# Autodesk Inventor assembly: Lift - Main Drive Sprocket
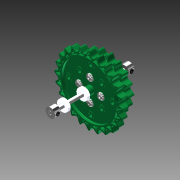
[picture p0: Inventor's stored thumbnail of the model, 180x180]
Saved by Autodesk Inventor 2012 (Build 160160000, 160)
## iProperties
Created: 2011-09-10
Part Number: Lift - Main Drive Sprocket
Document SubType Name: Assembly
Designer: Wade
Author: Wade
## Documents named in this file (9)
- C:\Users\Wade\Documents\1103 Robot - CAD Assembly\Lift - Main Drive Sprocket.iam
- C:\Users\Wade\Documents\24C VEX CAD Files\Drive Shafts\Drive Shaft (Square Bar) 3.625''.ipt
- C:\Users\Wade\Documents\24C VEX CAD Files\Gears & Pulleys\High Strength 24-Tooth Sprocket.ipt
- C:\Users\Wade\Documents\24C VEX CAD Files\Gears & Pulleys\High Strength 18-Tooth Sprocket.ipt
- C:\Users\Wade\Documents\1103 Robot - CAD Assembly\BEAM-0500.ipt
- C:\Users\Wade\Documents\24C VEX CAD Files\Other Parts\Shaft Collar (with Set Screw Installed).ipt
- C:\Users\Wade\Documents\24C VEX CAD Files\Washers & Spacers\Spacer (Nylon), 0.125''.ipt
- C:\Users\Wade\Documents\24C VEX CAD Files\Washers & Spacers\Spacer (Nylon), 0.250''.ipt
- C:\Users\Wade\Documents\24C VEX CAD Files\Screws & Nuts\Screw 8-32 x 0.375''-Silver.ipt
## Components (20 placed, 8 different names)
1. Drive Shaft (Square Bar) 3.625'':1 — Mate:1, Mate:2, Flush:1, Flush:2, Flush:4
2. High Strength 24-Tooth Sprocket:1 — Mate:1, Mate:2, Mate:3, Mate:4, Mate:5, Mate:6, Mate:7, Mate:8, Mate:9, Mate:10, Mate:11, Mate:22, Mate:23, Mate:24, Mate:25, Mate:26, Mate:27, Mate:28, Mate:29, Mate:31, Mate:33, Mate:35, Mate:36, Mate:37
3. High Strength 18-Tooth Sprocket:1 — Mate:11, Mate:12, Mate:13, Mate:14, Mate:15, Mate:16, Mate:17, Mate:18, Mate:19, Mate:20, Mate:21, Mate:30, Mate:32, Mate:34
4. BEAM-0500:1 — Mate:3, Mate:8, Mate:12, Mate:13
5. BEAM-0500:2 — Mate:5, Mate:10
6. BEAM-0500:3 — Mate:6, Mate:7
7. BEAM-0500:4 — Mate:4, Mate:9
8. Shaft Collar (with Set Screw Installed):1 — Mate:30, Flush:1, Flush:2, Flush:3, Mate:32
9. Shaft Collar (with Set Screw Installed):2 — Flush:3, Mate:31, Flush:4, Mate:38
10. Spacer (Nylon), 0.125'':1 — Mate:35, Mate:36
11. Spacer (Nylon), 0.125'':2 — Mate:37, Mate:38
12. Spacer (Nylon), 0.250'':1 — Mate:33, Mate:34
13. Screw 8-32 x 0.375''-Silver:1 — Mate:17, Mate:19
14. Screw 8-32 x 0.375''-Silver:2 — Mate:14, Mate:21
15. Screw 8-32 x 0.375''-Silver:3 — Mate:15, Mate:20
16. Screw 8-32 x 0.375''-Silver:4 — Mate:16, Mate:18
17. Screw 8-32 x 0.375''-Silver:5 — Mate:23, Mate:26
18. Screw 8-32 x 0.375''-Silver:6 — Mate:25, Mate:28
19. Screw 8-32 x 0.375''-Silver:7 — Mate:24, Mate:27
20. Screw 8-32 x 0.375''-Silver:8 — Mate:22, Mate:29
## Relationships (42: Mate 38, Flush 4)
- Mate:1: Drive Shaft (Square Bar) 3.625'':1 ↔ High Strength 24-Tooth Sprocket:1
- Mate:2: Drive Shaft (Square Bar) 3.625'':1 ↔ High Strength 24-Tooth Sprocket:1
- Mate:3: High Strength 24-Tooth Sprocket:1 ↔ BEAM-0500:1
- Mate:4: High Strength 24-Tooth Sprocket:1 ↔ BEAM-0500:4
- Mate:5: High Strength 24-Tooth Sprocket:1 ↔ BEAM-0500:2
- Mate:6: High Strength 24-Tooth Sprocket:1 ↔ BEAM-0500:3
- Mate:7: High Strength 24-Tooth Sprocket:1 ↔ BEAM-0500:3
- Mate:8: High Strength 24-Tooth Sprocket:1 ↔ BEAM-0500:1
- Mate:9: High Strength 24-Tooth Sprocket:1 ↔ BEAM-0500:4
- Mate:10: High Strength 24-Tooth Sprocket:1 ↔ BEAM-0500:2
- Mate:11: High Strength 24-Tooth Sprocket:1 ↔ High Strength 18-Tooth Sprocket:1
- Mate:12: High Strength 18-Tooth Sprocket:1 ↔ BEAM-0500:1
- Mate:13: High Strength 18-Tooth Sprocket:1 ↔ BEAM-0500:1
- Mate:14: High Strength 18-Tooth Sprocket:1 ↔ Screw 8-32 x 0.375''-Silver:2
- Mate:15: High Strength 18-Tooth Sprocket:1 ↔ Screw 8-32 x 0.375''-Silver:3
- Mate:16: High Strength 18-Tooth Sprocket:1 ↔ Screw 8-32 x 0.375''-Silver:4
- Mate:17: High Strength 18-Tooth Sprocket:1 ↔ Screw 8-32 x 0.375''-Silver:1
- Mate:18: High Strength 18-Tooth Sprocket:1 ↔ Screw 8-32 x 0.375''-Silver:4
- Mate:19: High Strength 18-Tooth Sprocket:1 ↔ Screw 8-32 x 0.375''-Silver:1
- Mate:20: High Strength 18-Tooth Sprocket:1 ↔ Screw 8-32 x 0.375''-Silver:3
- Mate:21: High Strength 18-Tooth Sprocket:1 ↔ Screw 8-32 x 0.375''-Silver:2
- Mate:22: High Strength 24-Tooth Sprocket:1 ↔ Screw 8-32 x 0.375''-Silver:8
- Mate:23: High Strength 24-Tooth Sprocket:1 ↔ Screw 8-32 x 0.375''-Silver:5
- Mate:24: High Strength 24-Tooth Sprocket:1 ↔ Screw 8-32 x 0.375''-Silver:7
- Mate:25: High Strength 24-Tooth Sprocket:1 ↔ Screw 8-32 x 0.375''-Silver:6
- Mate:26: High Strength 24-Tooth Sprocket:1 ↔ Screw 8-32 x 0.375''-Silver:5
- Mate:27: High Strength 24-Tooth Sprocket:1 ↔ Screw 8-32 x 0.375''-Silver:7
- Mate:28: High Strength 24-Tooth Sprocket:1 ↔ Screw 8-32 x 0.375''-Silver:6
- Mate:29: High Strength 24-Tooth Sprocket:1 ↔ Screw 8-32 x 0.375''-Silver:8
- Mate:30: High Strength 18-Tooth Sprocket:1 ↔ Shaft Collar (with Set Screw Installed):1
- Flush:1: Drive Shaft (Square Bar) 3.625'':1 ↔ Shaft Collar (with Set Screw Installed):1
- Flush:2: Drive Shaft (Square Bar) 3.625'':1 ↔ Shaft Collar (with Set Screw Installed):1
- Flush:3: Shaft Collar (with Set Screw Installed):1 ↔ Shaft Collar (with Set Screw Installed):2
- Mate:31: High Strength 24-Tooth Sprocket:1 ↔ Shaft Collar (with Set Screw Installed):2
- Flush:4: Drive Shaft (Square Bar) 3.625'':1 ↔ Shaft Collar (with Set Screw Installed):2
- Mate:32 (13.8684 mm): High Strength 18-Tooth Sprocket:1 ↔ Shaft Collar (with Set Screw Installed):1
- Mate:33: High Strength 24-Tooth Sprocket:1 ↔ Spacer (Nylon), 0.250'':1
- Mate:34: High Strength 18-Tooth Sprocket:1 ↔ Spacer (Nylon), 0.250'':1
- Mate:35: High Strength 24-Tooth Sprocket:1 ↔ Spacer (Nylon), 0.125'':1
- Mate:36: High Strength 24-Tooth Sprocket:1 ↔ Spacer (Nylon), 0.125'':1
- Mate:37: High Strength 24-Tooth Sprocket:1 ↔ Spacer (Nylon), 0.125'':2
- Mate:38 (7.5184 mm): Shaft Collar (with Set Screw Installed):2 ↔ Spacer (Nylon), 0.125'':2
